# Autodesk Inventor assembly: Assembly
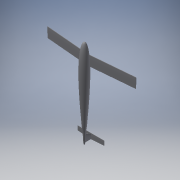
[picture p0: Inventor's stored thumbnail of the model, 180x180]
Saved by Autodesk Inventor 2019 (Build 230136000, 136)
## iProperties
Created: 2019-04-06
Part Number: Assembly
Document SubType Name: Assembly
Designer: albaa
Mass: 287.278 g
Surface Area: 32441.8 cm^2
Volume: 9575.95 cm^3
Density: 0.03 g/cm^3
Author: albaa
## Documents named in this file (5)
- C:\Users\albaa\Google Drive\McGill OneDrive\McGill\Courses\13_WINTER 2019\MECH 532\Project\REPO_mech532-project\CAD\Assembly.iam
- C:\Users\albaa\Google Drive\McGill OneDrive\McGill\Courses\13_WINTER 2019\MECH 532\Project\REPO_mech532-project\CAD\fuselage.ipt
- C:\Users\albaa\Google Drive\McGill OneDrive\McGill\Courses\13_WINTER 2019\MECH 532\Project\REPO_mech532-project\CAD\hTail_wing.ipt
- C:\Users\albaa\Google Drive\McGill OneDrive\McGill\Courses\13_WINTER 2019\MECH 532\Project\REPO_mech532-project\CAD\main_wing.ipt
- C:\Users\albaa\Google Drive\McGill OneDrive\McGill\Courses\13_WINTER 2019\MECH 532\Project\REPO_mech532-project\CAD\vTail_wing.ipt
## Components (4 placed, 4 different names)
1. fuselage:1 — Flush:1, Flush:2, Mate:1, Mate:2, Flush:7, Flush:10
2. hTail_wing:1 — Flush:5, Flush:6, Mate:2
3. main_wing:1 — Mate:1, Mate:3, Flush:11
4. vTail_wing:1 — Flush:7, Flush:8, Flush:9
## Relationships (12: Flush 9, Mate 3)
- Flush:1: fuselage:1
- Flush:2: fuselage:1
- Mate:1 (-500 mm): fuselage:1 ↔ main_wing:1
- Flush:5: hTail_wing:1
- Flush:6 (-150 mm): hTail_wing:1
- Mate:2: fuselage:1 ↔ hTail_wing:1
- Flush:7: fuselage:1 ↔ vTail_wing:1
- Flush:8: vTail_wing:1
- Flush:9: vTail_wing:1
- Flush:10: fuselage:1
- Mate:3 (80 mm): main_wing:1
- Flush:11: main_wing:1
